# Autodesk Inventor assembly: MainModule
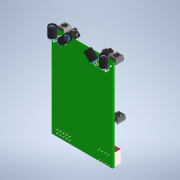
[picture p0: Inventor's stored thumbnail of the model, 180x180]
Saved by Autodesk Inventor 2021 (Build 250183000, 183)
## iProperties
Created: 2021-05-14
Part Number: MainModule
Document SubType Name: Assembly
Designer: ermoz
Author: ermoz
## Documents named in this file (7)
- D:\Moje Wyczyny\My_Poor_Projects\Sneak100_MiniSumo\minisumo-sneak100\mechanics\ElectricElements\MainModule.iam
- D:\Moje Wyczyny\My_Poor_Projects\Sneak100_MiniSumo\minisumo-sneak100\mechanics\ElectricElements\MainBoard.ipt
- D:\Moje Wyczyny\My_Poor_Projects\Sneak100_MiniSumo\minisumo-sneak100\mechanics\PreMadeParts\IDC_10_pin_connector.ipt
- D:\Moje Wyczyny\My_Poor_Projects\Sneak100_MiniSumo\minisumo-sneak100\mechanics\PreMadeParts\TSOP4838.ipt
- D:\Moje Wyczyny\My_Poor_Projects\Sneak100_MiniSumo\minisumo-sneak100\mechanics\PreMadeParts\STM32F303RE_LQFP64.ipt
- D:\Moje Wyczyny\My_Poor_Projects\Sneak100_MiniSumo\minisumo-sneak100\mechanics\PreMadeParts\IR_TSAL6400.ipt
- D:\Moje Wyczyny\My_Poor_Projects\Sneak100_MiniSumo\minisumo-sneak100\mechanics\PreMadeParts\Dip_switch_4.ipt
## Components (13 placed, 6 different names)
1. MainBoard:1 — Mate:1, Mate:2, Mate:3, Angle:1, Angle:2, Mate:5, Mate:6, Mate:7, Mate:8, Tangent:1, Tangent:2, Mate:9, Mate:10
2. IDC_10_pin_connector:1 — Mate:1
3. STM32F303RE_LQFP64:1 — Mate:3
4. IR_TSAL6400:1 — Mate:5, Flush:4, Tangent:1
5. IR_TSAL6400:2 — Mate:7
6. IR_TSAL6400:3 — Mate:8
7. IR_TSAL6400:4 — Mate:6, Flush:4, Tangent:2
8. TSOP4838:1 — Flush:5, Mate:10
9. TSOP4838:2 — Flush:2, Angle:2
10. TSOP4838:3 — Flush:2, Flush:3, Angle:1
11. TSOP4838:4 — Flush:3, Mate:9, Flush:5
12. TSOP4838:5
13. Dip_switch_4:1 — Mate:2
## Relationships (17: Mate 9, Flush 4, Angle 2, Tangent 2)
- Mate:1: MainBoard:1 ↔ IDC_10_pin_connector:1
- Mate:2: MainBoard:1 ↔ Dip_switch_4:1
- Mate:3: MainBoard:1 ↔ STM32F303RE_LQFP64:1
- Flush:2: TSOP4838:2 ↔ TSOP4838:3
- Flush:3: TSOP4838:3 ↔ TSOP4838:4
- Angle:1 (45 deg): MainBoard:1 ↔ TSOP4838:3
- Angle:2 (45 deg): MainBoard:1 ↔ TSOP4838:2
- Mate:5 (-2 mm): MainBoard:1 ↔ IR_TSAL6400:1
- Mate:6 (-2 mm): MainBoard:1 ↔ IR_TSAL6400:4
- Flush:4: IR_TSAL6400:1 ↔ IR_TSAL6400:4
- Mate:7 (-2 mm): MainBoard:1 ↔ IR_TSAL6400:2
- Mate:8 (-2 mm): MainBoard:1 ↔ IR_TSAL6400:3
- Tangent:1 (1 mm): MainBoard:1 ↔ IR_TSAL6400:1
- Tangent:2 (1 mm): MainBoard:1 ↔ IR_TSAL6400:4
- Mate:9: MainBoard:1 ↔ TSOP4838:4
- Flush:5: TSOP4838:1 ↔ TSOP4838:4
- Mate:10: MainBoard:1 ↔ TSOP4838:1
